# Autodesk Inventor assembly: Coupler top regular + pulleys
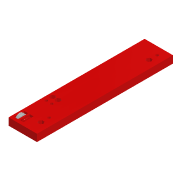
[picture p0: Inventor's stored thumbnail of the model, 180x180]
Saved by Autodesk Inventor 2020 (Build 240168000, 168)
## iProperties
Created: 2019-11-17
Part Number: Coupler top regular + pulleys
Document SubType Name: Assembly
Designer: ball
Author: ball
## Documents named in this file (5)
- C:\FTC\FTC8863CAD\2019 Robot\Delivery\Coupler top regular + pulleys.iam
- C:\FTC\FTC8863CAD\2019 Robot\Delivery\Coupler top regular.ipt
- C:\FTC\FTC8863CAD\2019 Robot\Delivery\plastic pulley deep u.ipt
- C:\FTC\FTC8863CAD\RevRobotics\REV-41-1368 pulley.ipt
- C:\FTC\FTC8863CAD\StepLibraries\Screws\M3 x 20 HEX HEAD CAP SCREW.ipt
## Components (4 placed, 4 different names)
1. Coupler top regular:1 — Mate:1, Mate:2, Mate:3, Mate:4, Mate:5, Mate:6
2. plastic pulley deep u:1 — Mate:1, Mate:2
3. REV-41-1368 pulley:1 — Mate:3, Mate:4
4. M3 x 20 HEX HEAD CAP SCREW:1 — Mate:5, Mate:6
## Relationships (6: Mate 6)
- Mate:1: Coupler top regular:1 ↔ plastic pulley deep u:1
- Mate:2: Coupler top regular:1 ↔ plastic pulley deep u:1
- Mate:3: Coupler top regular:1 ↔ REV-41-1368 pulley:1
- Mate:4: Coupler top regular:1 ↔ REV-41-1368 pulley:1
- Mate:5: Coupler top regular:1 ↔ M3 x 20 HEX HEAD CAP SCREW:1
- Mate:6: Coupler top regular:1 ↔ M3 x 20 HEX HEAD CAP SCREW:1
